# Autodesk Inventor assembly: Tiger.349c8af2-8c75-4afe-83c1-161ed9b79777
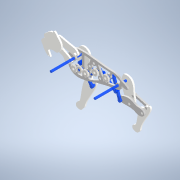
[picture p0: Inventor's stored thumbnail of the model, 180x180]
Saved by Autodesk Inventor 2022 (Build 260153000, 153)
## iProperties
Created: 2022-01-29
Part Number: Tiger.349c8af2-8c75-4afe-83c1-161ed9b79777
Document SubType Name: Assembly
Designer: Administrator
Title: Tiger.349c8af2-8c75-4afe-83c1-161ed9b79777 v1
Author: Administrator
## Documents named in this file (25)
- C:\Users\br4ch\M-and-Ms\Final project\Cyber Tiger\Inventor\Tiger.iam
- C:\Users\br4ch\M-and-Ms\Final project\Cyber Tiger\Inventor\Component9.ipt
- C:\Users\br4ch\M-and-Ms\Final project\Cyber Tiger\Inventor\Component16.ipt
- C:\Users\br4ch\M-and-Ms\Final project\Cyber Tiger\Inventor\Component18.ipt
- C:\Users\br4ch\M-and-Ms\Final project\Cyber Tiger\Inventor\Component19.ipt
- C:\Users\br4ch\M-and-Ms\Final project\Cyber Tiger\Inventor\Component20.ipt
- C:\Users\br4ch\M-and-Ms\Final project\Cyber Tiger\Inventor\Component25.ipt
- C:\Users\br4ch\M-and-Ms\Final project\Cyber Tiger\Inventor\Component26.ipt
- C:\Users\br4ch\M-and-Ms\Final project\Cyber Tiger\Inventor\Component27.ipt
- C:\Users\br4ch\M-and-Ms\Final project\Cyber Tiger\Inventor\Component28.ipt
- C:\Users\br4ch\M-and-Ms\Final project\Cyber Tiger\Inventor\Component29.ipt
- C:\Users\br4ch\M-and-Ms\Final project\Cyber Tiger\Inventor\Component30.ipt
- C:\Users\br4ch\M-and-Ms\Final project\Cyber Tiger\Inventor\Component31.ipt
- C:\Users\br4ch\M-and-Ms\Final project\Cyber Tiger\Inventor\Component32.ipt
- C:\Users\br4ch\M-and-Ms\Final project\Cyber Tiger\Inventor\Component33.ipt
- C:\Users\br4ch\M-and-Ms\Final project\Cyber Tiger\Inventor\Component34.ipt
- C:\Users\br4ch\M-and-Ms\Final project\Cyber Tiger\Inventor\Component35.ipt
- C:\Users\br4ch\M-and-Ms\Final project\Cyber Tiger\Inventor\Component36.ipt
- C:\Users\br4ch\M-and-Ms\Final project\Cyber Tiger\Inventor\Component37.ipt
- C:\Users\br4ch\M-and-Ms\Final project\Cyber Tiger\Inventor\Component38.ipt
- C:\Users\br4ch\M-and-Ms\Final project\Cyber Tiger\Inventor\Component39.ipt
- C:\Users\br4ch\M-and-Ms\Final project\Cyber Tiger\Inventor\Component40.ipt
- C:\Users\br4ch\M-and-Ms\Final project\Cyber Tiger\Inventor\Component41.ipt
- C:\Users\br4ch\M-and-Ms\Final project\Cyber Tiger\Inventor\Tiger\Design Accelerator\front gears3.iam
- C:\Users\br4ch\M-and-Ms\Final project\Cyber Tiger\Inventor\Tiger\Design Accelerator\front gears4.iam
## Components (30 placed, 23 different names)
1. Component40:1 — Rotational:41, Rigid:9, Rotational:42
2. Component41:1 — Rigid:7, Rigid:10
3. Component9:4 — Rotational:17, Cylindrical:2
4. Component16:3 — Rotational:14, Cylindrical:1
5. Component18:3 — Angle:2, Rotational:2, Rotational:3
6. Component19:3 — Rotational:3, Mate:15, Tangent:1, Symmetry:1
7. Component20:3 — Rotational:2, Rotational:4
8. Component25:3 — Rotational:13, Rotational:15
9. Component27:3 — Rotational:7, Rotational:10, Rotational:11
10. Component26:4 — Mate:15, Tangent:1, Rotational:4, Rotational:5, Rotational:6, Rotational:8, Cylindrical:1, Cylindrical:2, Rotational:19, Symmetry:1, Rotational:41, Rotational:42
11. Component37:3 — Rotational:18, Rigid:5, Rotational:5
12. Component29:3 — Rotational:6, Rotational:7, Rigid:3
13. Component31:3 — Rotational:8, Rotational:9, Rigid:6
14. Component39:3 — Rotational:9, Rotational:10
15. Component33:3 — Rotational:11, Rotational:12, Rotational:16
16. Component35:3 — Rotational:12, Rotational:13, Rotational:14
17. Component36:3 — Rotational:15, Rotational:16
18. Component34:3 — Rotational:17, Rotational:22
19. Component38:3 — Rotational:18, Rotational:21, Rotational:23
20. Component32:3 — Rotational:20, Rotational:21
21. Component28:3 — Rotational:19, Rotational:20, Rigid:7
22. Component30:3 — Rotational:22, Rotational:23
23. Component41:3 — Rigid:6, Rigid:11
24. Component41:4 — Rigid:3, Rigid:44
25. Component41:5 — Rigid:5, Rigid:8
26. front gears:1 [sub-assembly] — Rigid:8, Rotation:1
27. front gears:2 [sub-assembly] — Rigid:9, Rotation:1, Rotation:2
28. front gears:3 [sub-assembly] — Rigid:10, Rotation:2, Rotation:4
29. front gears:4 [sub-assembly] — Rigid:11, Rotation:3, Rotation:4
30. front gears:5 [sub-assembly] — Rigid:44, Rotation:3
## Relationships (43: RevoluteJoint 24, WeldJoint 9, RelateRotation 4, CylindricalJoint 2, Angle 1, Mate 1, Tangent 1, Symmetry 1)
- Angle:2 (0 deg): Component18:3
- Rotational:2 [RevoluteJoint]: Component18:3 ↔ Component20:3
- Rotational:3 [RevoluteJoint]: Component18:3 ↔ Component19:3
- Mate:15: Component19:3 ↔ Component26:4
- Tangent:1: Component19:3 ↔ Component26:4
- Rotational:4 [RevoluteJoint]: Component20:3 ↔ Component26:4
- Rotational:5 [RevoluteJoint]: Component26:4 ↔ Component37:3
- Rotational:6 [RevoluteJoint]: Component26:4 ↔ Component29:3
- Rotational:8 [RevoluteJoint]: Component26:4 ↔ Component31:3
- Rotational:7 [RevoluteJoint]: Component27:3 ↔ Component29:3
- Rotational:9 [RevoluteJoint]: Component31:3 ↔ Component39:3
- Rotational:10 [RevoluteJoint]: Component27:3 ↔ Component39:3
- Rotational:11 [RevoluteJoint]: Component27:3 ↔ Component33:3
- Rotational:12 [RevoluteJoint]: Component33:3 ↔ Component35:3
- Rotational:13 [RevoluteJoint]: Component25:3 ↔ Component35:3
- Rotational:14 [RevoluteJoint]: Component16:3 ↔ Component35:3
- Cylindrical:1: Component16:3 ↔ Component26:4
- Rotational:15 [RevoluteJoint]: Component25:3 ↔ Component36:3
- Rotational:16 [RevoluteJoint]: Component33:3 ↔ Component36:3
- Rotational:17 [RevoluteJoint]: Component9:4 ↔ Component34:3
- Cylindrical:2: Component9:4 ↔ Component26:4
- Rotational:18 [RevoluteJoint]: Component37:3 ↔ Component38:3
- Rotational:19 [RevoluteJoint]: Component26:4 ↔ Component28:3
- Rotational:20 [RevoluteJoint]: Component32:3 ↔ Component28:3
- Rotational:21 [RevoluteJoint]: Component38:3 ↔ Component32:3
- Rotational:22 [RevoluteJoint]: Component34:3 ↔ Component30:3
- Rotational:23 [RevoluteJoint]: Component38:3 ↔ Component30:3
- Symmetry:1: Component19:3 ↔ Component26:4
- Rigid:3 [WeldJoint]: Component29:3 ↔ Component41:4
- Rotational:41 [RevoluteJoint]: Component40:1 ↔ Component26:4
- Rigid:5 [WeldJoint]: Component37:3 ↔ Component41:5
- Rigid:6 [WeldJoint]: Component31:3 ↔ Component41:3
- Rigid:7 [WeldJoint]: Component41:1 ↔ Component28:3
- Rigid:8 [WeldJoint]: Component41:5 ↔ front gears:1
- Rigid:9 [WeldJoint]: Component40:1 ↔ front gears:2
- Rigid:10 [WeldJoint]: Component41:1 ↔ front gears:3
- Rotational:42 [RevoluteJoint]: Component40:1 ↔ Component26:4
- Rotation:1 [RelateRotation] (1 ul): front gears:1 ↔ front gears:2
- Rotation:2 [RelateRotation] (1 ul): front gears:2 ↔ front gears:3
- Rigid:11 [WeldJoint]: Component41:3 ↔ front gears:4
- Rigid:44 [WeldJoint]: Component41:4 ↔ front gears:5
- Rotation:3 [RelateRotation] (1 ul): front gears:4 ↔ front gears:5
- Rotation:4 [RelateRotation] (1 ul): front gears:3 ↔ front gears:4
## Named parameters: R = 6.5 mm, thickness = 5 mm, width = 6.5 mm, R1 = 9 mm
